# Autodesk Inventor assembly: ASY Мешалка
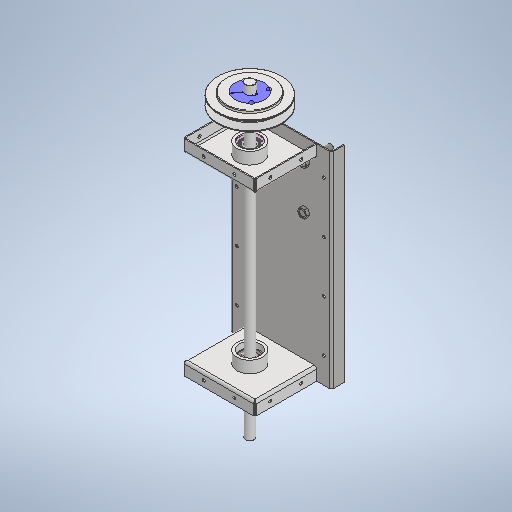
[picture p0: Inventor's stored thumbnail of the model, 512x512]
Saved by Autodesk Inventor 2025 (Build 290162010, 162A)
## iProperties
Created: 2024-04-09
Part Number: ASY Мешалка
Document SubType Name: Assembly
Designer: pokla
Stock Number: ASY Мешалка
Author: pokla
## Documents named in this file (12)
- C:\Users\pokla\Documents\Inventor\Gusev_Meshalka\ASY Мешалка\ASY Мешалка.iam
- C:\Users\pokla\Documents\Inventor\Gusev_Meshalka\ASY Мешалка\SKF B7203 BE.ipt
- C:\Users\pokla\Documents\Inventor\Gusev_Meshalka\ASY Мешалка\CSN 02 9401 - G 17x40x7 - NBR.ipt
- C:\Users\pokla\Documents\Inventor\Gusev_Meshalka\ASY Мешалка\Шкив 119 мм.ipt
- Шкив 119 мм.ipt
- C:\Users\pokla\Documents\Inventor\Gusev_Meshalka\ASY Мешалка\Втулка для шкива.ipt
- C:\Users\pokla\Documents\Inventor\Gusev_Meshalka\ASY Мешалка\ANSI B 27.7M - 3AMI-17.ipt
- C:\Users\pokla\Documents\Inventor\Gusev_Meshalka\ASY Мешалка\ANSI B 27.7M - 3BMI-40.ipt
- C:\Users\pokla\Documents\Inventor\Gusev_Meshalka\ASY Мешалка\Корпус.iam
- C:\Users\pokla\Documents\Inventor\Gusev_Meshalka\ASY Мешалка\Седло для сальника.ipt
- C:\Users\pokla\Documents\Inventor\Gusev_Meshalka\ASY Мешалка\Седло для подшипника.ipt
- C:\Users\pokla\Documents\Inventor\Gusev_Meshalka\ASY Мешалка\Shaft1.ipt
## Components (15 placed, 10 different names)
1. SKF B7203 BE.ipt:1 — Rigid:3
2. SKF B7203 BE.ipt:2 — Rigid:6
3. CSN 02 9401 - G 17x40x7 - NBR.ipt:1 — Rigid:12
4. CSN 02 9401 - G 17x40x7 - NBR.ipt:2 — Rigid:13
5. Шкив 119 мм.ipt:1 — Rotational:2
6. Втулка для шкива.ipt:1 — Rigid:17, Rotational:2
7. ANSI B 27.7M - 3AMI-17.ipt:1 — Rigid:15
8. ANSI B 27.7M - 3BMI-40.ipt:1 — Rigid:7
9. ANSI B 27.7M - 3BMI-40.ipt:2 — Rigid:2
10. Корпус.iam:1 [sub-assembly] — Flush:1, Flush:2, Flush:3, Rigid:4, Rigid:5
11. Седло для сальника.ipt:1 — Rigid:4, Rigid:6, Rigid:7, Rigid:9, Rigid:12, Rigid:14
12. Седло для подшипника.ipt:1 — Rigid:2, Rigid:3, Rigid:5, Rigid:13
13. ANSI B 27.7M - 3BMI-40.ipt:3 — Rigid:9
14. ANSI B 27.7M - 3AMI-17.ipt:2 — Rigid:16
15. Shaft:1 — Rigid:14, Rigid:15, Rigid:16, Rigid:17
## Relationships (17: WeldJoint 13, Flush 3, RevoluteJoint 1)
- Flush:1: Корпус.iam:1
- Flush:2: Корпус.iam:1
- Flush:3: Корпус.iam:1
- Rigid:2 [WeldJoint]: ANSI B 27.7M - 3BMI-40.ipt:2 ↔ Седло для подшипника.ipt:1
- Rigid:3 [WeldJoint]: SKF B7203 BE.ipt:1 ↔ Седло для подшипника.ipt:1
- Rigid:4 [WeldJoint] (23 mm): Корпус.iam:1 ↔ Седло для сальника.ipt:1
- Rigid:5 [WeldJoint] (23 mm): Корпус.iam:1 ↔ Седло для подшипника.ipt:1
- Rigid:6 [WeldJoint]: SKF B7203 BE.ipt:2 ↔ Седло для сальника.ipt:1
- Rigid:7 [WeldJoint]: ANSI B 27.7M - 3BMI-40.ipt:1 ↔ Седло для сальника.ipt:1
- Rigid:9 [WeldJoint]: Седло для сальника.ipt:1 ↔ ANSI B 27.7M - 3BMI-40.ipt:3
- Rigid:12 [WeldJoint]: CSN 02 9401 - G 17x40x7 - NBR.ipt:1 ↔ Седло для сальника.ipt:1
- Rigid:13 [WeldJoint]: CSN 02 9401 - G 17x40x7 - NBR.ipt:2 ↔ Седло для подшипника.ipt:1
- Rigid:14 [WeldJoint] (20 mm): Седло для сальника.ipt:1 ↔ Shaft:1
- Rigid:15 [WeldJoint]: ANSI B 27.7M - 3AMI-17.ipt:1 ↔ Shaft:1
- Rigid:16 [WeldJoint]: ANSI B 27.7M - 3AMI-17.ipt:2 ↔ Shaft:1
- Rigid:17 [WeldJoint] (-16.3 mm): Втулка для шкива.ipt:1 ↔ Shaft:1
- Rotational:2 [RevoluteJoint]: Шкив 119 мм.ipt:1 ↔ Втулка для шкива.ipt:1
